# Autodesk Inventor assembly: Base
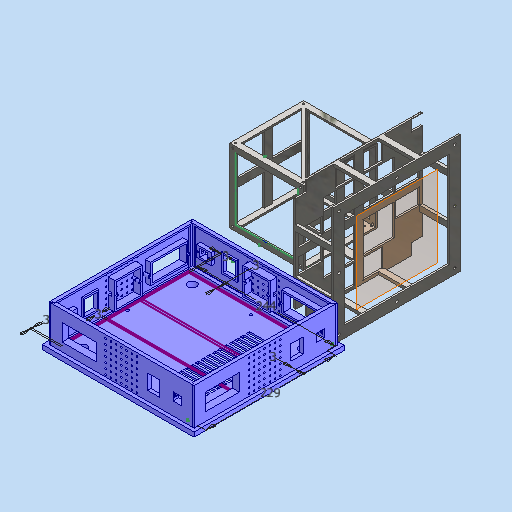
[picture p0: Inventor's stored thumbnail of the model, 512x512]
Saved by Autodesk Inventor 2027 (Build 310192000, 192)
## iProperties
Created: 2026-10-07
Part Number: Base
Document SubType Name: Assembly
Designer: alex
Author: alex
## Documents named in this file (5)
- C:\Users\alex\Documents\BocetoDigital\Base.iam
- C:\Users\alex\Documents\BocetoDigital\BaseCara.ipt
- C:\Users\alex\Documents\BocetoDigital\BaseTras.ipt
- C:\Users\alex\Documents\BocetoDigital\Base.ipt
- C:\Users\alex\Documents\BocetoDigital\EsctructuraCaja.ipt
## Components (6 placed, 4 different names)
1. BaseCara:1 — Coincidencia:1, Nivelación:1, Nivelación:2, Coincidencia:2, Coincidencia:3, Nivelación:3, Coincidencia:4, Coincidencia:9
2. BaseCara:2 — Coincidencia:1, Nivelación:1, Nivelación:2, Coincidencia:2, Coincidencia:5, Coincidencia:6, Coincidencia:8, Coincidencia:10
3. BaseCara:3 — Coincidencia:3, Nivelación:3, Coincidencia:4, Coincidencia:7
4. BaseTras:1 — Coincidencia:5, Coincidencia:6, Coincidencia:7
5. Base:1 — Coincidencia:8, Coincidencia:9, Coincidencia:10
6. EsctructuraCaja:1
## Relationships (13: Mate 10, Flush 3)
- Coincidencia:1 [Mate]: BaseCara:1 ↔ BaseCara:2
- Nivelación:1 [Flush]: BaseCara:1 ↔ BaseCara:2
- Nivelación:2 [Flush]: BaseCara:1 ↔ BaseCara:2
- Coincidencia:2 [Mate]: BaseCara:1 ↔ BaseCara:2
- Coincidencia:3 [Mate]: BaseCara:1 ↔ BaseCara:3
- Nivelación:3 [Flush]: BaseCara:1 ↔ BaseCara:3
- Coincidencia:4 [Mate]: BaseCara:1 ↔ BaseCara:3
- Coincidencia:5 [Mate]: BaseCara:2 ↔ BaseTras:1
- Coincidencia:6 [Mate]: BaseCara:2 ↔ BaseTras:1
- Coincidencia:7 [Mate]: BaseCara:3 ↔ BaseTras:1
- Coincidencia:8 [Mate]: BaseCara:2 ↔ Base:1
- Coincidencia:9 [Mate]: BaseCara:1 ↔ Base:1
- Coincidencia:10 [Mate]: BaseCara:2 ↔ Base:1
